# Autodesk Inventor assembly: S2_Yaxis_Rail_500
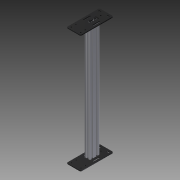
[picture p0: Inventor's stored thumbnail of the model, 180x180]
Saved by Autodesk Inventor 2014 (Build 180170000, 170)
## iProperties
Created: 2013-09-18
Part Number: S2_Yaxis_Rail_500
Document SubType Name: Assembly
Designer: Edward
Author: Edward
## Documents named in this file (6)
- C:\Users\Edward\Documents\Vault\Designs\Shapeoko_v2\v2_final\assemblies\S2_Yaxis_Rail_500.iam
- C:\Users\Edward\Documents\Vault\Designs\Shapeoko_v2\v2_final\26028-01.ipt
- C:\Users\Edward\Documents\Vault\Designs\Shapeoko_v2\v2_final\25286-02.ipt
- C:\Users\Edward\Documents\Vault\Designs\Shapeoko_v2\v2_final\25287-02.ipt
- C:\Users\Edward\Documents\Vault\Designs\Shapeoko_v2\v2_final\belt_clip_assembly.iam
- C:\Users\Edward\Documents\Vault\Designs\Shapeoko_v2\v2_final\25142-XX500.ipt
## Components (13 placed, 5 different names)
1. 25142-XX500:1
2. 26028-01:1
3. 26028-01:2
4. 25286-02:1
5. 25287-02:1
6. 25286-02:2
7. 25287-02:2
8. 25286-02:3
9. 25287-02:3
10. 25286-02:4
11. 25287-02:4
12. belt_clip_assembly:1 [sub-assembly]
13. belt_clip_assembly:2 [sub-assembly]
## Relationships (18: Insert 10, Mate 4, Angle 2, Flush 2)
- [Insert]: 25142-XX500:1 ↔ 26028-01:2
- [Insert]: 25142-XX500:1 ↔ 26028-01:1
- [Angle] (0 deg): 26028-01:1 ↔ 26028-01:2
- [Angle] (0 deg): 25142-XX500:1 ↔ 26028-01:2
- [Insert]: 25286-02:1 ↔ 25287-02:1
- [Insert]: 25286-02:2 ↔ 25287-02:2
- [Insert] (3.4163 mm): 25142-XX500:1 ↔ 25287-02:2
- [Insert] (3.4163 mm): 25142-XX500:1 ↔ 25287-02:1
- [Insert]: 25286-02:3 ↔ 25287-02:3
- [Insert]: 25286-02:4 ↔ 25287-02:4
- [Insert]: 26028-01:1 ↔ 25287-02:4
- [Insert] (3.4163 mm): 25142-XX500:1 ↔ 25287-02:3
- [Mate]: 25142-XX500:1 ↔ belt_clip_assembly:2
- [Mate]: 26028-01:1 ↔ belt_clip_assembly:2
- [Flush] (3 mm): 25142-XX500:1 ↔ belt_clip_assembly:2
- [Mate]: 25142-XX500:1 ↔ belt_clip_assembly:1
- [Flush] (3 mm): 25142-XX500:1 ↔ belt_clip_assembly:1
- [Mate]: 26028-01:2 ↔ belt_clip_assembly:1
## Named parameters: d52_d51 = 0 mm, d79_d51 = 0 mm, d80_d51 = 0 mm, d16_d18 = 0 mm
